# Autodesk Inventor assembly: Final Assembly
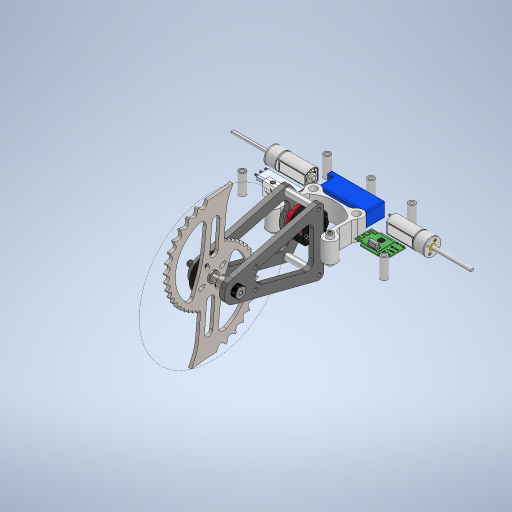
[picture p0: Inventor's stored thumbnail of the model, 512x512]
Saved by Autodesk Inventor 2023.1 (Build 271208000, 208)
## iProperties
Created: 2022-08-25
Part Number: Final Assembly
Document SubType Name: Assembly
Designer: Nathan Cai
Mass: 266.713 g
Surface Area: 638.287 cm^2
Volume: 73.7735 cm^3
Density: 3.6153 g/cm^3
Author: Nathan Cai
## Documents named in this file (10)
- E:\Documents\Inventor\3rd Lawelle - V0.1\Final Assembly.iam
- E:\Documents\Inventor\3rd Lawelle - V0.1\Weapon Assembly.iam
- E:\Documents\Inventor\3rd Lawelle - V0.1\Malenki-Nano_2020 (1) v1.ipt
- E:\Documents\Inventor\3rd Lawelle - V0.1\BL20A.ipt
- E:\Documents\Inventor\3rd Lawelle - V0.1\Battery-G-2S-300 Lipo.ipt
- E:\Documents\Inventor\3rd Lawelle - V0.1\Fingertech Power Switch\Fingertech Mini Power Switch.iam
- E:\Documents\Inventor\3rd Lawelle - V0.1\FT SilverSpark 33\FingerTech_Silver_Spark_223350 (1).ipt
- E:\Documents\Inventor\3rd Lawelle - V0.1\Spacer 1in.ipt
- E:\Documents\Inventor\3rd Lawelle - V0.1\92510A447_Aluminum Unthreaded Spacer.ipt
- E:\Documents\Inventor\3rd Lawelle - V0.1\Chassis.ipt
## Components (15 placed, 9 different names)
1. Weapon Assembly:1 [sub-assembly]
2. Malenki-Nano_2020 (1) v1:1
3. BL20A:1
4. Battery-G-2S-300 Lipo:1
5. Fingertech Mini Power Switch:1 [sub-assembly]
6. FingerTech_Silver_Spark_223350 (1):1 — Mate:1, Flush:1
7. FingerTech_Silver_Spark_223350 (1):2 — Mate:1, Flush:1
8. Spacer 1in:1 — Mate:2, Flush:3
9. Spacer 1in:2 — Mate:3, Flush:2
10. 92510A447_Aluminum Unthreaded Spacer:1
11. 92510A447_Aluminum Unthreaded Spacer:3
12. 92510A447_Aluminum Unthreaded Spacer:5
13. 92510A447_Aluminum Unthreaded Spacer:6
14. 92510A447_Aluminum Unthreaded Spacer:7
15. Chassis:1 — Mate:2, Mate:3, Flush:2, Flush:3
## Relationships (6: Mate 3, Flush 3)
- Mate:1: FingerTech_Silver_Spark_223350 (1):1 ↔ FingerTech_Silver_Spark_223350 (1):2
- Flush:1: FingerTech_Silver_Spark_223350 (1):1 ↔ FingerTech_Silver_Spark_223350 (1):2
- Mate:2: Spacer 1in:1 ↔ Chassis:1
- Mate:3: Spacer 1in:2 ↔ Chassis:1
- Flush:2 (-3.175 mm): Spacer 1in:2 ↔ Chassis:1
- Flush:3 (-3.175 mm): Spacer 1in:1 ↔ Chassis:1
